# Autodesk Inventor assembly: bay con 12 mk2
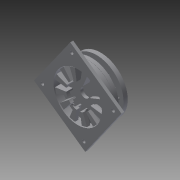
[picture p0: Inventor's stored thumbnail of the model, 180x180]
Saved by Autodesk Inventor 2015 (Build 190159000, 159)
## iProperties
Created: 2014-10-24
Part Number: bay con 12 mk2
Document SubType Name: Assembly
Designer: ericd_000
Author: ericd_000
## Documents named in this file (7)
- C:\Users\ericd_000\Dropbox\GitHub\initial_cad\eric_cad\bay con 12 mk2.iam
- C:\Users\ericd_000\Dropbox\GitHub\initial_cad\eric_cad\bayonet container 12.ipt
- C:\Users\ericd_000\Dropbox\GitHub\initial_cad\eric_cad\inner bayonet connector 12.ipt
- C:\Users\ericd_000\Dropbox\GitHub\initial_cad\eric_cad\bay container 12 bottom.ipt
- C:\Users\ericd_000\Dropbox\GitHub\initial_cad\eric_cad\Imported Components\M3 25MM\M3 25MM.ipt
- C:\Users\ericd_000\Dropbox\GitHub\initial_cad\eric_cad\Imported Components\m3 nut\m3 nut.ipt
- C:\Users\ericd_000\Dropbox\GitHub\initial_cad\eric_cad\Imported Components\8mm length spring\8mm length spring.ipt
## Components (8 placed, 6 different names)
1. bayonet container 12:1 — Cylindrical:1, Cylindrical:2, Cylindrical:10, Mate:5, Cylindrical:11, Mate:6
2. inner bayonet connector 12:1 — Cylindrical:1, Cylindrical:2
3. bay container 12 bottom:1 — Mate:3, Mate:4, Cylindrical:9, Cylindrical:12, Cylindrical:13
4. m3 nut:1 — Mate:4, Cylindrical:14
5. m3 nut:2 — Mate:3, Cylindrical:15
6. 8mm length spring:1 — Cylindrical:9
7. M3 25MM:1 — Cylindrical:10, Mate:5, Cylindrical:13, Cylindrical:14
8. M3 25MM:2 — Cylindrical:11, Mate:6, Cylindrical:12, Cylindrical:15
## Relationships (13: CylindricalJoint 9, Mate 4)
- Cylindrical:1: bayonet container 12:1 ↔ inner bayonet connector 12:1
- Cylindrical:2: bayonet container 12:1 ↔ inner bayonet connector 12:1
- Mate:3 (0.4 mm): bay container 12 bottom:1 ↔ m3 nut:2
- Mate:4 (0.4 mm): bay container 12 bottom:1 ↔ m3 nut:1
- Cylindrical:9: bay container 12 bottom:1 ↔ 8mm length spring:1
- Cylindrical:10: bayonet container 12:1 ↔ M3 25MM:1
- Mate:5: bayonet container 12:1 ↔ M3 25MM:1
- Cylindrical:11: bayonet container 12:1 ↔ M3 25MM:2
- Mate:6: bayonet container 12:1 ↔ M3 25MM:2
- Cylindrical:12: bay container 12 bottom:1 ↔ M3 25MM:2
- Cylindrical:13: bay container 12 bottom:1 ↔ M3 25MM:1
- Cylindrical:14: m3 nut:1 ↔ M3 25MM:1
- Cylindrical:15: m3 nut:2 ↔ M3 25MM:2
